# Autodesk Inventor assembly: Figure hinge
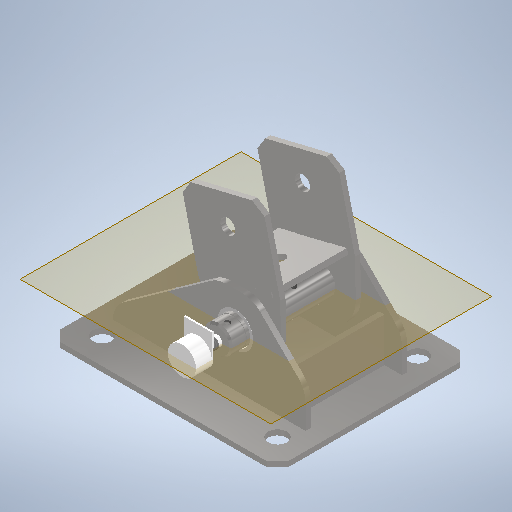
[picture p0: Inventor's stored thumbnail of the model, 512x512]
Saved by Autodesk Inventor 2025.2 (Build 292293000, 293)
## iProperties
Created: 2025-05-27
Part Number: Figure hinge
Document SubType Name: Assembly
Designer: Caspe
Author: Caspe
## Documents named in this file (5)
- C:\Users\Caspe\Documents\Semester 8\Project\Anomaly_Detection\Mechanical_Project\Inventor_project\Figure hinge.iam
- C:\Users\Caspe\Documents\Semester 8\Project\Anomaly_Detection\Mechanical_Project\Inventor_project\bottom_hinge_pot.iam
- C:\Users\Caspe\Documents\Semester 8\Project\Anomaly_Detection\Mechanical_Project\Inventor_project\A_beam_end_mount.iam
- C:\Users\Caspe\Documents\Inventor\Content Center Files\R2025\en-US\DIN 915\DIN 915 - M3 x 5.ipt
- C:\Users\Caspe\Documents\Semester 8\Project\Anomaly_Detection\Mechanical_Project\Inventor_project\bushing.ipt
## Components (4 placed, 4 different names)
1. bottom_hinge_pot:1 [sub-assembly] — Mate:1, Mate:2, Mate:3, Insert:1, Flush:1
2. A_beam_end_mount:1 [sub-assembly] — Mate:1, Mate:2
3. DIN 915 M3 x 5:1 — Mate:3
4. bushing:1 — Insert:1
## Relationships (5: Mate 3, Insert 1, Flush 1)
- Mate:1: bottom_hinge_pot:1 ↔ A_beam_end_mount:1
- Mate:2 (3 mm): bottom_hinge_pot:1 ↔ A_beam_end_mount:1
- Mate:3: bottom_hinge_pot:1 ↔ DIN 915 M3 x 5:1
- Insert:1: bottom_hinge_pot:1 ↔ bushing:1
- Flush:1 (29.75 mm): bottom_hinge_pot:1
